# Autodesk Inventor assembly: arm shaft SUB
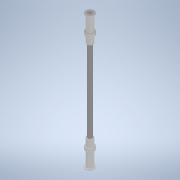
[picture p0: Inventor's stored thumbnail of the model, 180x180]
Saved by Autodesk Inventor 2021 (Build 250183000, 183)
## iProperties
Created: 2021-03-29
Part Number: arm shaft SUB
Document SubType Name: Assembly
Designer: Work
Author: Work
## Documents named in this file (4)
- C:\Users\Work\OneDrive - Brookhaven National Laboratory\Daniels, William intern HPR station\Arm\arm shaft SUB.iam
- C:\Users\Work\OneDrive - Brookhaven National Laboratory\Daniels, William intern HPR station\Arm\arm shaft.ipt
- C:\Users\Work\OneDrive - Brookhaven National Laboratory\Daniels, William intern HPR station\Arm\59575K710_DRY-RUNNING SLEEVE BEARING WITH METAL SHELL.ipt
- C:\Users\Work\OneDrive - Brookhaven National Laboratory\Daniels, William intern HPR station\Arm\arm shaft spacer.ipt
## Components (9 placed, 3 different names)
1. arm shaft:1 — Rigid:1, Rigid:3
2. 59575K710_DRY-RUNNING SLEEVE BEARING WITH METAL SHELL:1 — Rigid:3, Rigid:4
3. 59575K710_DRY-RUNNING SLEEVE BEARING WITH METAL SHELL:2 — Rigid:4, Rigid:7
4. 59575K710_DRY-RUNNING SLEEVE BEARING WITH METAL SHELL:3 — Rigid:8
5. 59575K710_DRY-RUNNING SLEEVE BEARING WITH METAL SHELL:4 — Rigid:1, Rigid:2
6. 59575K710_DRY-RUNNING SLEEVE BEARING WITH METAL SHELL:5 — Rigid:2, Rigid:5
7. 59575K710_DRY-RUNNING SLEEVE BEARING WITH METAL SHELL:6 — Rigid:6
8. arm shaft spacer:1 — Rigid:7, Rigid:8
9. arm shaft spacer:2 — Rigid:5, Rigid:6
## Relationships (8: WeldJoint 8)
- Rigid:1 [WeldJoint]: arm shaft:1 ↔ 59575K710_DRY-RUNNING SLEEVE BEARING WITH METAL SHELL:4
- Rigid:2 [WeldJoint]: 59575K710_DRY-RUNNING SLEEVE BEARING WITH METAL SHELL:4 ↔ 59575K710_DRY-RUNNING SLEEVE BEARING WITH METAL SHELL:5
- Rigid:3 [WeldJoint]: arm shaft:1 ↔ 59575K710_DRY-RUNNING SLEEVE BEARING WITH METAL SHELL:1
- Rigid:4 [WeldJoint]: 59575K710_DRY-RUNNING SLEEVE BEARING WITH METAL SHELL:1 ↔ 59575K710_DRY-RUNNING SLEEVE BEARING WITH METAL SHELL:2
- Rigid:5 [WeldJoint]: 59575K710_DRY-RUNNING SLEEVE BEARING WITH METAL SHELL:5 ↔ arm shaft spacer:2
- Rigid:6 [WeldJoint]: 59575K710_DRY-RUNNING SLEEVE BEARING WITH METAL SHELL:6 ↔ arm shaft spacer:2
- Rigid:7 [WeldJoint]: 59575K710_DRY-RUNNING SLEEVE BEARING WITH METAL SHELL:2 ↔ arm shaft spacer:1
- Rigid:8 [WeldJoint]: 59575K710_DRY-RUNNING SLEEVE BEARING WITH METAL SHELL:3 ↔ arm shaft spacer:1
